# Autodesk Inventor assembly: wire guidance
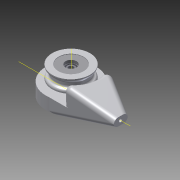
[picture p0: Inventor's stored thumbnail of the model, 180x180]
Saved by Autodesk Inventor 2013 (Build 170138000, 138)
## iProperties
Created: 2012-11-22
Part Number: wire guidance
Document SubType Name: Assembly
Designer: Nico
Author: Nico
## Documents named in this file (7)
- D:\Documents\Inventor\Coil winder\IAM files\wire guidance.iam
- D:\Documents\Inventor\Coil winder\IPT files\wire guide.ipt
- D:\Documents\Inventor\Content Center Files\R2013\en-US\ISO 1224 (I) M\ISO 1224 - 39 - 3 x 8 x 4.ipt
- D:\Documents\Inventor\Coil winder\IPT files\Bearring cap 8mm.ipt
- D:\Documents\Inventor\Coil winder\IAM files\guide wheel.iam
- D:\Documents\Inventor\Coil winder\IPT files\Nut M3 nickel plated.ipt
- D:\Documents\Inventor\Coil winder\IPT files\Nut M3 Torque nickel plated.ipt
## Components (6 placed, 6 different names)
1. wire guide:1 — Mate:14, Mate:15, Mate:16, Mate:17
2. ISO 1224 (I) (Metric) 39 - 3 x 8 x 4:1 — Mate:15, Mate:16, Mate:20
3. Bearring cap 8mm:1 — Mate:9, Mate:17
4. guide wheel:1 [sub-assembly] — Mate:9, Mate:10, Mate:11, Mate:14
5. Nut M3 Torque nickel plated:1 — Mate:19, Mate:20, Mate:21
6. Nut M3 nickel plated:2 — Mate:10, Mate:11, Mate:19, Mate:21
## Relationships (10: Mate 10)
- Mate:9: Bearring cap 8mm:1 ↔ guide wheel:1
- Mate:10: guide wheel:1 ↔ Nut M3 nickel plated:2
- Mate:11: guide wheel:1 ↔ Nut M3 nickel plated:2
- Mate:14: wire guide:1 ↔ guide wheel:1
- Mate:15: wire guide:1 ↔ ISO 1224 (I) (Metric) 39 - 3 x 8 x 4:1
- Mate:16: wire guide:1 ↔ ISO 1224 (I) (Metric) 39 - 3 x 8 x 4:1
- Mate:17: wire guide:1 ↔ Bearring cap 8mm:1
- Mate:19: Nut M3 Torque nickel plated:1 ↔ Nut M3 nickel plated:2
- Mate:20: ISO 1224 (I) (Metric) 39 - 3 x 8 x 4:1 ↔ Nut M3 Torque nickel plated:1
- Mate:21: Nut M3 Torque nickel plated:1 ↔ Nut M3 nickel plated:2
